# Autodesk Inventor assembly: assembly with new 5 inch shaft transmission'
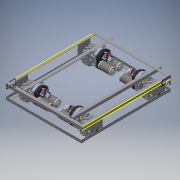
[picture p0: Inventor's stored thumbnail of the model, 180x180]
Saved by Autodesk Inventor 2016 SP2 (Build 200236200, 236)
## iProperties
Created: 2018-02-06
Part Number: assembly with new 5 inch shaft transmission'
Document SubType Name: Assembly
Designer: CAD
Author: CAD
## Documents named in this file (6)
- C:\Users\CAD\Documents\GitHub\FIRST-ROBOTICS-2018-5436-CAD\Robot\Chassis\assembly with new 5 inch shaft transmission'.iam
- C:\Users\CAD\Documents\GitHub\FIRST-ROBOTICS-2018-5436-CAD\Robot\Chassis\Transmission parts\Transmission w 5 inch shaft and bracket assembly.iam
- C:\Users\CAD\Documents\GitHub\FIRST-ROBOTICS-2018-5436-CAD\Robot\Chassis\27.5 L.ipt
- C:\Users\CAD\Documents\GitHub\FIRST-ROBOTICS-2018-5436-CAD\Robot\Chassis\27.5 Top L.ipt
- C:\Users\CAD\Documents\GitHub\FIRST-ROBOTICS-2018-5436-CAD\Robot\Chassis\32.25 Top L.ipt
- C:\Users\CAD\Documents\GitHub\FIRST-ROBOTICS-2018-5436-CAD\Robot\Chassis\32.25 L.ipt
## Components (14 placed, 5 different names)
1. Transmission w 5 inch shaft and bracket assembly:1 [sub-assembly] — Mate:4, Mate:10, Flush:7
2. Transmission w 5 inch shaft and bracket assembly:2 [sub-assembly] — Mate:3, Mate:9, Mate:15
3. Transmission w 5 inch shaft and bracket assembly:3 [sub-assembly] — Mate:2, Mate:6, Flush:6, Mate:8
4. Transmission w 5 inch shaft and bracket assembly:4 [sub-assembly] — Mate:1, Mate:5, Mate:7, Mate:13, Mate:14
5. 32.25 Top L:1 — Mate:5, Mate:6, Flush:6, Mate:7, Mate:8, Mate:18, Flush:11
6. 32.25 Top L:2 — Mate:9, Mate:10, Flush:7, Mate:16, Mate:17, Flush:10, Mate:21, Mate:22, Flush:15
7. 32.25 L:1 — Mate:3, Mate:4, Flush:5, Flush:12, Mate:19, Mate:20, Flush:13, Mate:23, Mate:24, Mate:25, Flush:16
8. 32.25 L:2 — Mate:1, Mate:2, Flush:5, Flush:12, Flush:14
9. 27.5 L:6 — Mate:16, Mate:17, Flush:10, Mate:18, Flush:11
10. 27.5 Top L:6 — Mate:19, Mate:20, Flush:13, Flush:14
11. 32.25 Top L:3 — Mate:13, Mate:14
12. 32.25 Top L:4 — Mate:15
13. 27.5 L:7 — Mate:21, Mate:22, Flush:15
14. 27.5 Top L:7 — Mate:23, Mate:24, Mate:25, Flush:16
## Relationships (33: Mate 23, Flush 10)
- Mate:1: Transmission w 5 inch shaft and bracket assembly:4 ↔ 32.25 L:2
- Mate:2: Transmission w 5 inch shaft and bracket assembly:3 ↔ 32.25 L:2
- Mate:3: Transmission w 5 inch shaft and bracket assembly:2 ↔ 32.25 L:1
- Mate:4: Transmission w 5 inch shaft and bracket assembly:1 ↔ 32.25 L:1
- Flush:5: 32.25 L:1 ↔ 32.25 L:2
- Mate:5: Transmission w 5 inch shaft and bracket assembly:4 ↔ 32.25 Top L:1
- Mate:6: Transmission w 5 inch shaft and bracket assembly:3 ↔ 32.25 Top L:1
- Flush:6 (-47.625 mm): Transmission w 5 inch shaft and bracket assembly:3 ↔ 32.25 Top L:1
- Mate:7: Transmission w 5 inch shaft and bracket assembly:4 ↔ 32.25 Top L:1
- Mate:8: Transmission w 5 inch shaft and bracket assembly:3 ↔ 32.25 Top L:1
- Mate:9: Transmission w 5 inch shaft and bracket assembly:2 ↔ 32.25 Top L:2
- Mate:10: Transmission w 5 inch shaft and bracket assembly:1 ↔ 32.25 Top L:2
- Flush:7 (47.625 mm): Transmission w 5 inch shaft and bracket assembly:1 ↔ 32.25 Top L:2
- Mate:13: Transmission w 5 inch shaft and bracket assembly:4 ↔ 32.25 Top L:3
- Mate:14: Transmission w 5 inch shaft and bracket assembly:4 ↔ 32.25 Top L:3
- Mate:15: Transmission w 5 inch shaft and bracket assembly:2 ↔ 32.25 Top L:4
- Mate:16: 32.25 Top L:2 ↔ 27.5 L:6
- Mate:17: 32.25 Top L:2 ↔ 27.5 L:6
- Flush:10: 32.25 Top L:2 ↔ 27.5 L:6
- Mate:18: 32.25 Top L:1 ↔ 27.5 L:6
- Flush:11: 32.25 Top L:1 ↔ 27.5 L:6
- Flush:12: 32.25 L:1 ↔ 32.25 L:2
- Mate:19: 32.25 L:1 ↔ 27.5 Top L:6
- Mate:20: 32.25 L:1 ↔ 27.5 Top L:6
- Flush:13: 32.25 L:1 ↔ 27.5 Top L:6
- Flush:14: 32.25 L:2 ↔ 27.5 Top L:6
- Mate:21: 32.25 Top L:2 ↔ 27.5 L:7
- Mate:22: 32.25 Top L:2 ↔ 27.5 L:7
- Flush:15: 32.25 Top L:2 ↔ 27.5 L:7
- Mate:23: 32.25 L:1 ↔ 27.5 Top L:7
- Mate:24: 32.25 L:1 ↔ 27.5 Top L:7
- Mate:25: 32.25 L:1 ↔ 27.5 Top L:7
- Flush:16: 32.25 L:1 ↔ 27.5 Top L:7
